# Autodesk Inventor assembly: MotorDC
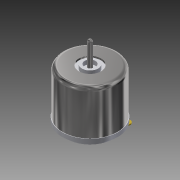
[picture p0: Inventor's stored thumbnail of the model, 180x180]
Saved by Autodesk Inventor 2013 (Build 170138000, 138)
## iProperties
Created: 2013-06-25
Part Number: MotorDC
Document SubType Name: Assembly
Designer: usuario
Author: usuario
## Documents named in this file (6)
- C:\Users\usuario\Desktop\MotorDC\MotorDC.iam
- C:\Users\usuario\Desktop\MotorDC\CajaMotor.ipt
- C:\Users\usuario\Desktop\MotorDC\TapaFrontal.ipt
- C:\Users\usuario\Desktop\MotorDC\TapaPosterior.ipt
- C:\Users\usuario\Desktop\MotorDC\EjeMotor.ipt
- C:\Users\usuario\Desktop\MotorDC\Conector.ipt
## Components (6 placed, 5 different names)
1. CajaMotor:1 — Insertar:1, Coincidencia:1, Insertar:2
2. TapaFrontal:1 — Insertar:1
3. TapaPosterior:1 — Coincidencia:1, Insertar:2, Coincidencia:2, Insertar:4, Insertar:5
4. EjeMotor:1 — Coincidencia:2
5. Conector:1 — Insertar:4
6. Conector:2 — Insertar:5
## Relationships (6: Insert 4, Mate 2)
- Insertar:1 (0.8 mm): CajaMotor:1 ↔ TapaFrontal:1
- Coincidencia:1 [Mate]: CajaMotor:1 ↔ TapaPosterior:1
- Insertar:2: CajaMotor:1 ↔ TapaPosterior:1
- Coincidencia:2 [Mate]: TapaPosterior:1 ↔ EjeMotor:1
- Insertar:4 (-4 mm): TapaPosterior:1 ↔ Conector:1
- Insertar:5 (-4 mm): TapaPosterior:1 ↔ Conector:2
